# Autodesk Inventor assembly: stylo assemblé
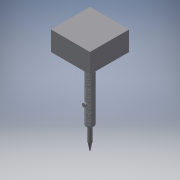
[picture p0: Inventor's stored thumbnail of the model, 180x180]
Saved by Autodesk Inventor 2017 (Build 210142000, 142)
## iProperties
Created: 2018-11-17
Part Number: stylo assemblé
Document SubType Name: Assembly
Designer: Antoine Blaud
Author: Antoine Blaud
## Documents named in this file (5)
- D:\Document\C\Arduino\project\pièces\petit\stylo assemblé.iam
- D:\Document\C\Arduino\project\pièces\petit\ressort.ipt
- D:\Document\C\Arduino\project\pièces\petit\stylo part1.ipt
- D:\Document\C\Arduino\project\pièces\petit\bout stylo.ipt
- D:\Document\C\Arduino\project\pièces\petit\contre poid.ipt
## Components (4 placed, 4 different names)
1. ressort:1 — Mate:1, Mate:2
2. stylo part1:1 — Mate:1, Mate:2, Mate:3, Angle:1, Mate:4, Mate:5, Mate:6
3. bout stylo:1 — Mate:3, Angle:1, Mate:4
4. contre poid:1 — Mate:5, Mate:6
## Relationships (7: Mate 6, Angle 1)
- Mate:1: ressort:1 ↔ stylo part1:1
- Mate:2: ressort:1 ↔ stylo part1:1
- Mate:3: stylo part1:1 ↔ bout stylo:1
- Angle:1 (180 deg): stylo part1:1 ↔ bout stylo:1
- Mate:4: stylo part1:1 ↔ bout stylo:1
- Mate:5: stylo part1:1 ↔ contre poid:1
- Mate:6: stylo part1:1 ↔ contre poid:1
